# Autodesk Inventor assembly: PneumaticWheel_am-0970
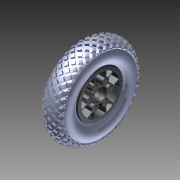
[picture p0: Inventor's stored thumbnail of the model, 180x180]
Saved by Autodesk Inventor 2013 (Build 170138000, 138)
## iProperties
Created: 2012-01-09
Part Number: PneumaticWheel_am-0970
Document SubType Name: Assembly
Designer: Nemo
Mass: 512.559 g
Surface Area: 2399.53 cm^2
Volume: 453.438 cm^3
Translation Standard: STEP AP214IS
FileName: Pneumatic Wheel.STEP
PreProcessor: SolidWorks 2010
PostProcessor: Build: 239, Release: 2011 RTM - Date: Wed 02/17/2010
Sent Units: inch
Uncertainty: 1e-05
Author: Nemo
## Documents named in this file (4)
- \\lmss\STUDENTS\Robotics\CAD Files\COTS Parts\Wheels\AndyMark Pneumatic Wheels\8in Pneumatic Wheel.iam
- \\lmss\STUDENTS\Robotics\CAD Files\COTS Parts\Wheels\AndyMark Pneumatic Wheels\Components\Tire.ipt
- \\lmss\STUDENTS\Robotics\CAD Files\COTS Parts\Wheels\AndyMark Pneumatic Wheels\Components\Valve.ipt
- \\lmss\STUDENTS\Robotics\CAD Files\COTS Parts\Wheels\AndyMark Pneumatic Wheels\Components\Pneumatic Hub.iam
## Components (3 placed, 3 different names)
1. Tire:1 — Angle:1, Mate:1, Angle:2, Mate:2, Mate:3, Mate:4
2. Valve:1
3. Pneumatic Hub:1 [sub-assembly]
## Relationships (6: Mate 4, Angle 2)
- Angle:1 (0 deg): Tire:1
- Mate:1: Tire:1
- Angle:2 (0 deg): Tire:1
- Mate:2: Tire:1
- Mate:3: Tire:1
- Mate:4: Tire:1
